# Autodesk Inventor assembly: Caseassembly
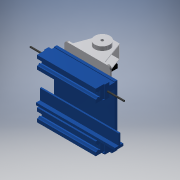
[picture p0: Inventor's stored thumbnail of the model, 180x180]
Saved by Autodesk Inventor 2016 (Build 200138000, 138)
## iProperties
Created: 2015-05-19
Part Number: Caseassembly
Document SubType Name: Assembly
Designer: Andy
Mass: 4028 g
Surface Area: 2840.2 cm^2
Volume: 1457.97 cm^3
Author: Andy
## Documents named in this file (4)
- C:\Users\jonathan\Desktop\Inverted Pendulum CAD\Track Assembly.iam
- C:\Users\jonathan\Desktop\Inverted Pendulum CAD\Track Casing.ipt
- C:\Users\jonathan\Desktop\Inverted Pendulum CAD\Track Encoder.ipt
- C:\Users\jonathan\Desktop\Inverted Pendulum CAD\Track Platform.ipt
## Components (3 placed, 3 different names)
1. Track Casing:1 — Mate:1, Mate:2, Angle:1, Mate:3, Flush:1, Flush:2
2. Track Encoder:1 — Mate:1, Mate:2, Angle:1
3. Track Platform:1 — Mate:3, Flush:1, Flush:2
## Relationships (6: Mate 3, Flush 2, Angle 1)
- Mate:1: Track Casing:1 ↔ Track Encoder:1
- Mate:2: Track Casing:1 ↔ Track Encoder:1
- Angle:1 (90 deg): Track Casing:1 ↔ Track Encoder:1
- Mate:3: Track Casing:1 ↔ Track Platform:1
- Flush:1 (150 mm): Track Casing:1 ↔ Track Platform:1
- Flush:2 (24.5 mm): Track Casing:1 ↔ Track Platform:1
